# Autodesk Inventor assembly: Octanis1_Rover_Rev04_Musk
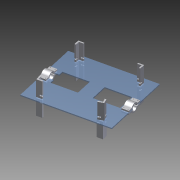
[picture p0: Inventor's stored thumbnail of the model, 180x180]
Saved by Autodesk Inventor 2014 SP1 (Build 180222100, 222)
## iProperties
Created: 2015-10-28
Part Number: Octanis1_Rover_Rev04_Musk
Document SubType Name: Assembly
Designer: Sam
Author: Sam
## Documents named in this file (7)
- C:\Users\Sam\Documents\GitHub\Octanis1-CAD\CAD_Rover_Rev04_Musk\Octanis1_Rover_Rev04_Musk.iam
- C:\Users\Sam\Documents\GitHub\Octanis1-CAD\CAD_Rover_Rev04_Musk\Imported Components\BasePlateInnerCornerPositioner\BasePlateInnerCornerPositioner.ipt
- C:\Users\Sam\Documents\GitHub\Octanis1-CAD\CAD_Rover_Rev04_Musk\Imported Components\BasePlate\BasePlate.ipt
- C:\Users\Sam\Documents\GitHub\Octanis1-CAD\CAD_Rover_Rev04_Musk\Imported Components\BasePlateInnerCornerPositioner\BasePlateInnerCornerPositioner_MIR.ipt
- C:\Users\Sam\Documents\GitHub\Octanis1-CAD\CAD_Rover_Rev04_Musk\Imported Components\BasePlateInnerCornerPositioner\BasePlateInnerCornerPositioner_MIR_CPY.ipt
- C:\Users\Sam\Documents\GitHub\Octanis1-CAD\CAD_Rover_Rev04_Musk\Imported Components\BasePlateInnerCornerPositioner\BasePlateInnerCornerPositioner_MIR_CPY_CPY.ipt
- C:\Users\Sam\Documents\GitHub\Octanis1-CAD\CAD_Rover_Rev04_Musk\Imported Components\PTFE_Tube_ScrewClamp\PTFE_Tube_ScrewClamp.ipt
## Components (13 placed, 6 different names)
1. BasePlateInnerCornerPositioner:2 — Rotational:3, Angle:3
2. BasePlateInnerCornerPositioner:5 — Rotational:10, Angle:7
3. BasePlateInnerCornerPositioner:6 — Rigid:2
4. BasePlateInnerCornerPositioner:7 — Angle:5, Rotational:7
5. BasePlate:1 — Rotational:3, Angle:3, Rigid:2, Rotational:6, Angle:4, Angle:5, Rotational:7, Angle:6, Rotational:9, Rotational:10, Angle:7, Rotational:11, Angle:8, Rotational:12, Mate:1, Mate:2, Flush:1, Mate:3
6. BasePlateInnerCornerPositioner_MIR:1 — Angle:6, Rotational:9
7. BasePlateInnerCornerPositioner_MIR_CPY:1 — Rotational:12
8. BasePlateInnerCornerPositioner_MIR_CPY_CPY:1 — Rotational:6, Angle:4
9. BasePlateInnerCornerPositioner_MIR_CPY:2 — Rotational:11, Angle:8
10. PTFE_Tube_ScrewClamp:1 — Flush:1, Mate:3, Rigid:4
11. PTFE_Tube_ScrewClamp:2 — Rigid:3
12. PTFE_Tube_ScrewClamp:3 — Mate:1, Mate:2, Rigid:3
13. PTFE_Tube_ScrewClamp:4 — Rigid:4
## Relationships (20: RevoluteJoint 7, Angle 6, WeldJoint 3, Mate 3, Flush 1)
- Rotational:3 [RevoluteJoint]: BasePlateInnerCornerPositioner:2 ↔ BasePlate:1
- Angle:3 (180 deg): BasePlateInnerCornerPositioner:2 ↔ BasePlate:1
- Rigid:2 [WeldJoint]: BasePlateInnerCornerPositioner:6 ↔ BasePlate:1
- Rotational:6 [RevoluteJoint]: BasePlate:1 ↔ BasePlateInnerCornerPositioner_MIR_CPY_CPY:1
- Angle:4 (0 deg): BasePlate:1 ↔ BasePlateInnerCornerPositioner_MIR_CPY_CPY:1
- Angle:5 (270 deg): BasePlateInnerCornerPositioner:7 ↔ BasePlate:1
- Rotational:7 [RevoluteJoint]: BasePlateInnerCornerPositioner:7 ↔ BasePlate:1
- Angle:6 (180 deg): BasePlate:1 ↔ BasePlateInnerCornerPositioner_MIR:1
- Rotational:9 [RevoluteJoint]: BasePlate:1 ↔ BasePlateInnerCornerPositioner_MIR:1
- Rotational:10 [RevoluteJoint]: BasePlateInnerCornerPositioner:5 ↔ BasePlate:1
- Angle:7 (270 deg): BasePlateInnerCornerPositioner:5 ↔ BasePlate:1
- Rotational:11 [RevoluteJoint]: BasePlate:1 ↔ BasePlateInnerCornerPositioner_MIR_CPY:2
- Angle:8 (180 deg): BasePlate:1 ↔ BasePlateInnerCornerPositioner_MIR_CPY:2
- Rotational:12 [RevoluteJoint]: BasePlate:1 ↔ BasePlateInnerCornerPositioner_MIR_CPY:1
- Mate:1: BasePlate:1 ↔ PTFE_Tube_ScrewClamp:3
- Mate:2: BasePlate:1 ↔ PTFE_Tube_ScrewClamp:3
- Rigid:3 [WeldJoint] (4 mm): PTFE_Tube_ScrewClamp:2 ↔ PTFE_Tube_ScrewClamp:3
- Flush:1: BasePlate:1 ↔ PTFE_Tube_ScrewClamp:1
- Mate:3: BasePlate:1 ↔ PTFE_Tube_ScrewClamp:1
- Rigid:4 [WeldJoint] (4 mm): PTFE_Tube_ScrewClamp:1 ↔ PTFE_Tube_ScrewClamp:4
